# Autodesk Inventor assembly: bottom plate assy
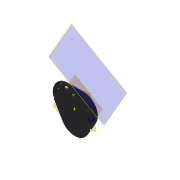
[picture p0: Inventor's stored thumbnail of the model, 180x180]
Saved by Autodesk Inventor 2016 (Build 200138000, 138)
## iProperties
Created: 2016-08-18
Part Number: bottom plate assy
Document SubType Name: Assembly
Designer: admin
Author: admin
## Documents named in this file (10)
- C:\Users\Juny\OneDrive - (주)에이팀벤처스\ateam\CL 3D프린터 사업- 설계 이준영\(((( delta 3D printer))))\20. 20190104 D3\1612 D3 3D modeling\bottom plate assy\bottom plate assy.iam
- C:\Users\Juny\OneDrive - (주)에이팀벤처스\ateam\CL 3D프린터 사업- 설계 이준영\(((( delta 3D printer))))\20. 20190104 D3\1612 D3 3D modeling\bottom plate assy\bed.ipt
- C:\Users\Juny\OneDrive - (주)에이팀벤처스\ateam\CL 3D프린터 사업- 설계 이준영\(((( delta 3D printer))))\20. 20190104 D3\1612 D3 3D modeling\bottom plate assy\bottom_plate.ipt
- C:\Users\Juny\OneDrive - (주)에이팀벤처스\ateam\CL 3D프린터 사업- 설계 이준영\(((( delta 3D printer))))\20. 20190104 D3\1612 D3 3D modeling\bottom plate assy\glass_plate.ipt
- C:\Users\Juny\OneDrive - (주)에이팀벤처스\ateam\CL 3D프린터 사업- 설계 이준영\(((( delta 3D printer))))\20. 20190104 D3\1612 D3 3D modeling\bottom plate assy\leveling_screw.ipt
- C:\Users\Juny\OneDrive - (주)에이팀벤처스\ateam\CL 3D프린터 사업- 설계 이준영\(((( delta 3D printer))))\20. 20190104 D3\1612 D3 3D modeling\bottom plate assy\leveling_spring.ipt
- C:\Users\Juny\OneDrive - (주)에이팀벤처스\ateam\CL 3D프린터 사업- 설계 이준영\(((( delta 3D printer))))\20. 20190104 D3\1612 D3 3D modeling\bottom plate assy\leveling_wheel.ipt
- C:\Users\Juny\OneDrive - (주)에이팀벤처스\ateam\CL 3D프린터 사업- 설계 이준영\(((( delta 3D printer))))\20. 20190104 D3\1612 D3 3D modeling\bottom plate assy\m3 5 Socket_Head.ipt
- C:\Users\Juny\OneDrive - (주)에이팀벤처스\ateam\CL 3D프린터 사업- 설계 이준영\(((( delta 3D printer))))\20. 20190104 D3\1612 D3 3D modeling\bottom plate assy\m8 hex_nut.ipt
- C:\Users\Juny\OneDrive - (주)에이팀벤처스\ateam\CL 3D프린터 사업- 설계 이준영\(((( delta 3D printer))))\20. 20190104 D3\1612 D3 3D modeling\bottom plate assy\bed clip 5.ipt
## Components (9 placed, 9 different names)
1. bed:1 — Mate:1, Rotational:7, Rotational:8, Rotational:9
2. bottom_plate:1 — Rotational:4, Rotational:5, Mate:1, Angle:3
3. glass_plate:1 — Rotational:8
4. leveling_spring:1 — Rotational:3
5. leveling_wheel:1 — Rotational:1, Rotational:5
6. m8 hex_nut:1 — Rotational:1
7. leveling_screw:1 — Rotational:3, Rotational:4, Angle:3
8. m3 5 Socket_Head:1 — Rotational:7
9. bed clip 5:2 — Rotational:9
## Relationships (9: RevoluteJoint 7, Mate 1, Angle 1)
- Rotational:1 [RevoluteJoint]: leveling_wheel:1 ↔ m8 hex_nut:1
- Rotational:3 [RevoluteJoint]: leveling_spring:1 ↔ leveling_screw:1
- Rotational:4 [RevoluteJoint] (-12 mm): bottom_plate:1 ↔ leveling_screw:1
- Rotational:5 [RevoluteJoint]: bottom_plate:1 ↔ leveling_wheel:1
- Mate:1: bed:1 ↔ bottom_plate:1
- Rotational:7 [RevoluteJoint]: bed:1 ↔ m3 5 Socket_Head:1
- Angle:3 (0 deg): bottom_plate:1 ↔ leveling_screw:1
- Rotational:8 [RevoluteJoint]: bed:1 ↔ glass_plate:1
- Rotational:9 [RevoluteJoint]: bed:1 ↔ bed clip 5:2
